# Autodesk Inventor assembly: Right Front Wheel with hub shaft and pulley
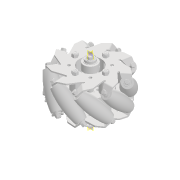
[picture p0: Inventor's stored thumbnail of the model, 180x180]
Saved by Autodesk Inventor 2020 (Build 240168000, 168)
## iProperties
Created: 2020-02-22
Part Number: Right Front Wheel with hub shaft and pulley
Document SubType Name: Assembly
Designer: ball
Author: ball
## Documents named in this file (7)
- C:\FTC\FTC8863CAD\2019 Robot\Mecanum Drive Train Metal\Right Front Wheel with hub shaft and pulley.iam
- C:\FTC\FTC8863CAD\2019 Robot\Mecanum Drive Train Metal\Right Front Wheel with hub.iam
- C:\FTC\FTC8863CAD\GoBilda\2102 Parts\2102-0008-0090.ipt
- C:\FTC\FTC8863CAD\GoBilda\3414 Parts\3414-4008-0016 assembly.iam
- C:\FTC\FTC8863CAD\GoBilda\1601 Parts\1601-0014-0008.ipt
- C:\FTC\FTC8863CAD\GoBilda\2807 Parts\2807-0811-0500.ipt
- C:\FTC\FTC8863CAD\GoBilda\2910 Parts\2910-1020-4008 assembly.ipt
## Components (7 placed, 6 different names)
1. Right Front Wheel with hub:1 [sub-assembly] — Mate:1, Mate:2, Mate:3
2. 2102-0008-0090:1 — Mate:1, Mate:2, Mate:4, Mate:5, Flush:2, Mate:6, Mate:7, Mate:9, Flush:3
3. 3414-4008-0016 assembly:1 [sub-assembly] — Mate:3, Mate:4, Mate:5, Mate:8
4. 1601-0014-0008:1 — Flush:2, Mate:6, Mate:11, Mate:12
5. 1601-0014-0008:2 — Mate:7, Mate:10, Flush:3
6. 2807-0811-0500:1 — Mate:8, Mate:9, Mate:10
7. 2910-1020-4008 assembly:1 — Mate:11, Mate:12
## Relationships (14: Mate 12, Flush 2)
- Mate:1: Right Front Wheel with hub:1 ↔ 2102-0008-0090:1
- Mate:2: Right Front Wheel with hub:1 ↔ 2102-0008-0090:1
- Mate:3: Right Front Wheel with hub:1 ↔ 3414-4008-0016 assembly:1
- Mate:4: 2102-0008-0090:1 ↔ 3414-4008-0016 assembly:1
- Mate:5: 2102-0008-0090:1 ↔ 3414-4008-0016 assembly:1
- Flush:2 (6.35 mm): 2102-0008-0090:1 ↔ 1601-0014-0008:1
- Mate:6: 2102-0008-0090:1 ↔ 1601-0014-0008:1
- Mate:7: 2102-0008-0090:1 ↔ 1601-0014-0008:2
- Mate:8: 3414-4008-0016 assembly:1 ↔ 2807-0811-0500:1
- Mate:9: 2102-0008-0090:1 ↔ 2807-0811-0500:1
- Mate:10: 1601-0014-0008:2 ↔ 2807-0811-0500:1
- Mate:11: 1601-0014-0008:1 ↔ 2910-1020-4008 assembly:1
- Mate:12: 1601-0014-0008:1 ↔ 2910-1020-4008 assembly:1
- Flush:3 (3.048 mm): 2102-0008-0090:1 ↔ 1601-0014-0008:2
